# Autodesk Inventor assembly: Montagem2
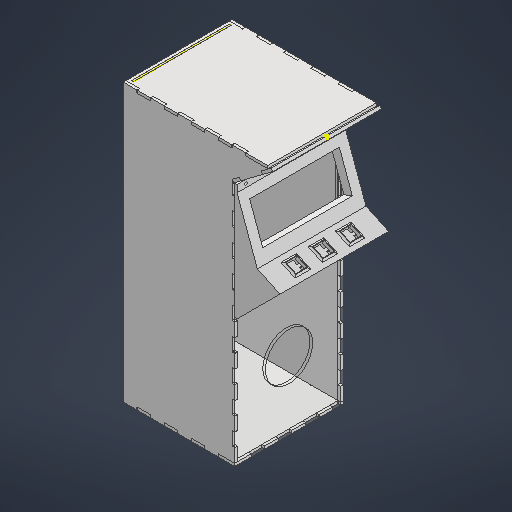
[picture p0: Inventor's stored thumbnail of the model, 512x512]
Saved by Autodesk Inventor 2026 (Build 300175050, 175E)
## iProperties
Created: 2025-08-08
Part Number: Montagem2
Document SubType Name: Assembly
Designer: EspacoMaker
Author: EspacoMaker
## Documents named in this file (8)
- C:\Users\EspacoMaker\Downloads\Cabine Acrilico - Particionado\Montagem2.iam
- C:\Users\EspacoMaker\Downloads\Cabine Acrilico - Particionado\Modelo Cabine - 3D.ipt
- C:\Users\EspacoMaker\Downloads\Cabine Acrilico - Particionado\NewVersions\frente.ipt
- C:\Users\EspacoMaker\Downloads\Cabine Acrilico - Particionado\NewVersions\side.ipt
- C:\Users\EspacoMaker\Downloads\Cabine Acrilico - Particionado\NewVersions\top.ipt
- C:\Users\EspacoMaker\Downloads\Cabine Acrilico - Particionado\NewVersions\Base.ipt
- C:\Users\EspacoMaker\Downloads\Cabine Acrilico - Particionado\NewVersions\top inclinado.ipt
- C:\Users\EspacoMaker\Downloads\Cabine Acrilico - Particionado\NewVersions\TAMPA.ipt
## Components (8 placed, 7 different names)
1. Modelo Cabine - 3D:1 — Coincidente:1, Alinhado:1, Alinhado:14
2. frente:1 — Coincidente:1, Alinhado:1, Alinhado:2, Alinhado:3, Alinhado:4, Alinhado:5, Alinhado:6, Alinhado:7, Alinhado:11, Alinhado:12, Alinhado:14
3. side:1 — Alinhado:2, Alinhado:3, Alinhado:4, Alinhado:8, Alinhado:9, Alinhado:10, Alinhado:13, Coincidente:2, Alinhado:15, Coincidente:3
4. side:2 — Alinhado:5, Alinhado:6, Alinhado:7
5. top:1 — Alinhado:8, Alinhado:9, Alinhado:10, Alinhado:16, Coincidente:4, Coincidente:5
6. Base:1 — Alinhado:11, Alinhado:12, Alinhado:13
7. top inclinado:1 — Coincidente:2, Alinhado:15, Coincidente:3
8. TAMPA:1 — Alinhado:16, Coincidente:4, Coincidente:5
## Relationships (21: Flush 16, Mate 5)
- Coincidente:1 [Mate]: Modelo Cabine - 3D:1 ↔ frente:1
- Alinhado:1 [Flush]: Modelo Cabine - 3D:1 ↔ frente:1
- Alinhado:2 [Flush]: frente:1 ↔ side:1
- Alinhado:3 [Flush]: frente:1 ↔ side:1
- Alinhado:4 [Flush]: frente:1 ↔ side:1
- Alinhado:5 [Flush]: frente:1 ↔ side:2
- Alinhado:6 [Flush]: frente:1 ↔ side:2
- Alinhado:7 [Flush]: frente:1 ↔ side:2
- Alinhado:8 [Flush]: side:1 ↔ top:1
- Alinhado:9 [Flush]: side:1 ↔ top:1
- Alinhado:10 [Flush]: side:1 ↔ top:1
- Alinhado:11 [Flush]: frente:1 ↔ Base:1
- Alinhado:12 [Flush]: frente:1 ↔ Base:1
- Alinhado:13 [Flush]: side:1 ↔ Base:1
- Alinhado:14 [Flush] (1 mm): Modelo Cabine - 3D:1 ↔ frente:1
- Coincidente:2 [Mate]: side:1 ↔ top inclinado:1
- Alinhado:15 [Flush]: side:1 ↔ top inclinado:1
- Coincidente:3 [Mate] (0.1 mm): side:1 ↔ top inclinado:1
- Alinhado:16 [Flush]: top:1 ↔ TAMPA:1
- Coincidente:4 [Mate] (0.1 mm): top:1 ↔ TAMPA:1
- Coincidente:5 [Mate] (0.1 mm): top:1 ↔ TAMPA:1
